# Autodesk Inventor assembly: hoverboard naked
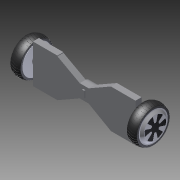
[picture p0: Inventor's stored thumbnail of the model, 180x180]
Saved by Autodesk Inventor 2014 SP2 (Build 180246200, 246)
## iProperties
Created: 2019-04-06
Part Number: hoverboard naked
Document SubType Name: Assembly
Designer: GauchoHP
Author: GauchoHP
## Documents named in this file (3)
- C:\Users\GauchoHP\Desktop\old_desktop\tosaerba\LAWNMOWER-ROBOT-from-Hoverboard-\LawnmowerMechanicalProject\3D PROJECT - INVENTOR 2014\hoverboard\hoverboard naked.iam
- C:\Users\GauchoHP\Desktop\old_desktop\tosaerba\LAWNMOWER-ROBOT-from-Hoverboard-\LawnmowerMechanicalProject\3D PROJECT - INVENTOR 2014\hoverboard\base\hoverboard plate.ipt
- C:\Users\GauchoHP\Desktop\old_desktop\tosaerba\LAWNMOWER-ROBOT-from-Hoverboard-\LawnmowerMechanicalProject\3D PROJECT - INVENTOR 2014\hoverboard\wheel\Motor, BLDC, Hoverboard Wheel, 6.5in.ipt
## Components (3 placed, 2 different names)
1. hoverboard plate:1 — Mate:1, Mate:2, Mate:3, Mate:4, Mate:5, Flush:1
2. Motor, BLDC, Hoverboard Wheel, 6.5in:1 — Mate:1, Mate:2, Mate:3
3. Motor, BLDC, Hoverboard Wheel, 6.5in:2 — Mate:4, Mate:5, Flush:1
## Relationships (6: Mate 5, Flush 1)
- Mate:1 (-14 mm): hoverboard plate:1 ↔ Motor, BLDC, Hoverboard Wheel, 6.5in:1
- Mate:2 (-22 mm): hoverboard plate:1 ↔ Motor, BLDC, Hoverboard Wheel, 6.5in:1
- Mate:3 (-61.5 mm): hoverboard plate:1 ↔ Motor, BLDC, Hoverboard Wheel, 6.5in:1
- Mate:4 (-14 mm): hoverboard plate:1 ↔ Motor, BLDC, Hoverboard Wheel, 6.5in:2
- Mate:5 (-22 mm): hoverboard plate:1 ↔ Motor, BLDC, Hoverboard Wheel, 6.5in:2
- Flush:1 (-61.5 mm): hoverboard plate:1 ↔ Motor, BLDC, Hoverboard Wheel, 6.5in:2
